# Autodesk Inventor assembly: Intake
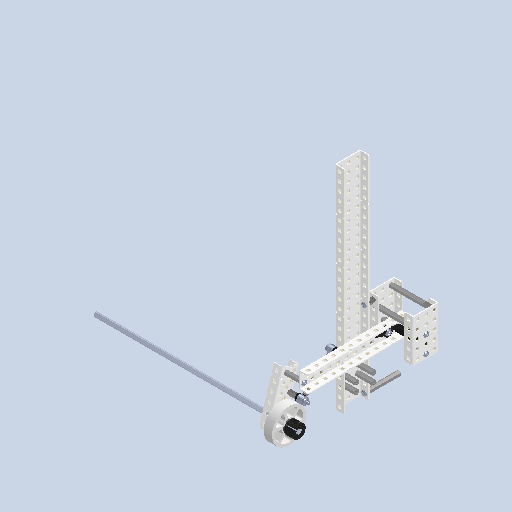
[picture p0: Inventor's stored thumbnail of the model, 512x512]
Saved by Autodesk Inventor 2023 (Build 270158000, 158)
## iProperties
Created: 2022-09-02
Part Number: Intake
Document SubType Name: Assembly
Designer: alex
Author: alex
## Documents named in this file (32)
- C:\Users\alex\Documents\GitHub\4067X_spin_up_cad\Mechanism\Intake.iam
- C:\Users\alex\Documents\GitHub\4067X_spin_up_cad\Library\Structure\C-Channels\Aluminum 1x3x1\Alu C 1x3x1x25.ipt
- C:\Users\alex\Documents\GitHub\4067X_spin_up_cad\Library\Structure\Standoff\Standoff 1.00.ipt
- C:\Users\alex\Documents\GitHub\4067X_spin_up_cad\Library\Structure\Standoff.ipt
- C:\Users\alex\Documents\GitHub\4067X_spin_up_cad\Library\Structure\Standoff\Standoff 2.00.ipt
- C:\Users\alex\Documents\GitHub\4067X_spin_up_cad\Library\Structure\Hardware\Screw Steel - Star\SScrew Star Smooth .290.ipt
- C:\Users\alex\Documents\GitHub\4067X_spin_up_cad\Library\Structure\Hardware\Screw Steel - Star.ipt
- C:\Users\alex\Documents\GitHub\4067X_spin_up_cad\Library\Structure\Standoff\Standoff .50.ipt
- C:\Users\alex\Documents\GitHub\4067X_spin_up_cad\Library\Structure\C-Channels\Aluminum 1x3x1\Alu C 1x3x1x5.ipt
- C:\Users\alex\Documents\GitHub\4067X_spin_up_cad\Library\Motion\Spacers\Spacer Nylon .375 OD.ipt
- C:\Users\alex\Documents\GitHub\4067X_spin_up_cad\Library\Motion\Spacers\Washer Teflon\TWasher .375 OD x .06250.ipt
- C:\Users\alex\Documents\GitHub\4067X_spin_up_cad\Library\Motion\Spacers\Washer Teflon.ipt
- C:\Users\alex\Documents\GitHub\4067X_spin_up_cad\Library\Structure\C-Channels\Aluminum 1x2x1\Alu C 1x2x1x6.ipt
- C:\Users\alex\Documents\GitHub\4067X_spin_up_cad\Library\Motion\Shaft HS\Shaft HS\Shaft HS 12.0 in.ipt
- C:\Users\alex\Documents\GitHub\4067X_spin_up_cad\Library\Motion\Shaft HS\Shaft HS.ipt
- C:\Users\alex\Documents\GitHub\4067X_spin_up_cad\Library\Motion\Spacers\Spacer Nylon .375 OD\NSpacer .375 OD x .125.ipt
- C:\Users\alex\Documents\GitHub\4067X_spin_up_cad\Library\Motion\Shaft Collar with Set Screw.ipt
- C:\Users\alex\Documents\GitHub\4067X_spin_up_cad\WithAdapter2Inch.iam
- C:\Users\alex\Documents\GitHub\4067X_spin_up_cad\Library\Motion\Shaft HS\HS Shaft Collar.ipt
- C:\Users\alex\Documents\GitHub\4067X_spin_up_cad\Library\Motion\Bearing Flat.ipt
- C:\Users\alex\Documents\GitHub\4067X_spin_up_cad\Library\Motion\Spacers\Spacer Nylon .375 OD\NSpacer .375 OD x .500.ipt
- C:\Users\alex\Documents\GitHub\4067X_spin_up_cad\Library\Motion\Spacers\Spacer Nylon .375 OD\NSpacer .375 OD x .375.ipt
- C:\Users\alex\Documents\GitHub\4067X_spin_up_cad\Library\Structure\Hardware\Screw Steel - Star\SScrew Star Smooth 1.250.ipt
- C:\Users\alex\Documents\GitHub\4067X_spin_up_cad\Library\Structure\Hardware\Nut Keps.ipt
- C:\Users\alex\Documents\GitHub\4067X_spin_up_cad\Library\Structure\Hardware\Screw Steel - Star\SScrew Star Smooth .625.ipt
- C:\Users\alex\Documents\GitHub\4067X_spin_up_cad\Library\Structure\Hardware\Screw Steel - Star\SScrew Star Threaded 2.500.ipt
- C:\Users\alex\Documents\GitHub\4067X_spin_up_cad\Library\Structure\C-Channels\Aluminum 1x2x1\Alu C 1x2x1x12.ipt
- C:\Users\alex\Documents\GitHub\4067X_spin_up_cad\Library\Motion\1-Post Bearing Flat Hex Retainer.ipt
- C:\Users\alex\Documents\GitHub\4067X_spin_up_cad\Library\Structure\Hardware\Screw Steel - Star\SScrew Star Smooth .375.ipt
- C:\Users\alex\Documents\GitHub\4067X_spin_up_cad\Library\Structure\Hardware\Nut Nylock.ipt
- C:\Users\alex\Documents\GitHub\4067X_spin_up_cad\Library\Structure\Hardware\Screw Steel - Star\SScrew Star Smooth .500.ipt
- C:\Users\alex\Documents\GitHub\4067X_spin_up_cad\Library\Structure\Hardware\Nut Thin Nylock.ipt
## Components (57 placed, 26 different names)
1. Alu C 1x3x1x25:1 — Insert:1, Insert:2, Insert:3, Insert:4, Insert:5, Insert:7, Insert:8, Insert:9, Insert:10, Insert:11, Insert:12, Insert:13, Insert:14, Insert:19
2. Standoff 1.00:1 — Insert:1
3. Standoff 1.00:2 — Insert:2
4. Standoff 1.00:3 — Insert:3
5. Standoff 1.00:4 — Insert:4
6. Standoff 2.00:5 — Insert:5
7. SScrew Star Smooth .290:1 — Insert:7
8. SScrew Star Smooth .290:2 — Insert:8
9. SScrew Star Smooth .290:3 — Insert:9
10. SScrew Star Smooth .290:4 — Insert:10
11. SScrew Star Smooth .290:5 — Insert:11
12. SScrew Star Smooth .290:6 — Insert:12
13. Standoff .50:6 — Insert:13, Insert:16
14. Alu C 1x3x1x5:1 — Insert:15, Insert:16, Insert:17, Insert:20, Insert:21, Insert:22, Insert:68, Insert:69, Insert:81, Insert:86
15. Standoff .50:7 — Insert:14, Insert:15
16. Standoff 2.00:8 — Insert:17, Insert:105
17. SScrew Star Smooth .290:7 — Insert:19
18. SScrew Star Smooth .290:8 — Insert:20
19. SScrew Star Smooth .290:9 — Insert:21
20. SScrew Star Smooth .290:10 — Insert:22
21. Alu C 1x2x1x6:1 — Mate:2, Mate:3, Insert:39, Insert:40, Mate:11, Insert:48, Insert:50
22. Shaft HS 12.0 in:1 — Mate:2, Mate:5, Mate:6, Mate:9, Mate:10, Flush:1
23. NSpacer .375 OD x .125:1 — Insert:34, Insert:73
24. Shaft Collar with Set Screw:1 — Insert:34, Mate:4, Mate:7, Insert:53
25. Shaft Collar with Set Screw:2 — Mate:3, Mate:4, Insert:35, Insert:49
26. WithAdapter2Inch:1 [sub-assembly] — Mate:5, Mate:6, Mate:8, Mate:11
27. Standoff 2.00:12 — Insert:35, Mate:7
28. Standoff .50:14 — Insert:38, Insert:39
29. NSpacer .375 OD x .125:2 — Insert:38
30. Standoff 1.00:15 — Insert:40, Insert:71
31. HS Shaft Collar:1 — Mate:8, Mate:9, Mate:10, Flush:1
32. SScrew Star Smooth 1.250:13 — Insert:48
33. Nut Keps:1 — Insert:49
34. SScrew Star Smooth .290:14 — Insert:50
35. SScrew Star Smooth .290:15 — Insert:72
36. SScrew Star Smooth .625:16 — Insert:74
37. Nut Keps:2 — Insert:53
38. SScrew Star Smooth .290:23 — Insert:68
39. Standoff 2.00:18 — Insert:69, Insert:106
40. Alu C 1x2x1x12:1 — Insert:71, Insert:72, Insert:73, Insert:74, Insert:83, Insert:102, Mate:12, Insert:103
41. Standoff .50:21 — Insert:81, Insert:82
42. TWasher .375 OD x .06250:1 — Insert:82, Insert:83
43. SScrew Star Threaded 2.500:25 — Insert:86
44. NSpacer .375 OD x .500:6 — Insert:111
45. 1-Post Bearing Flat Hex Retainer:1 — Insert:102, Mate:12, Insert:104
46. SScrew Star Smooth .375:30 — Insert:103
47. Nut Nylock:1 — Insert:104
48. Alu C 1x3x1x5:2 — Insert:107, Insert:108, Insert:109, Insert:110, Insert:113, Insert:114
49. Standoff .50:22 — Insert:105, Insert:107
50. Standoff .50:23 — Insert:106, Insert:108
51. Bearing Flat:3 — Insert:109, Insert:110, Insert:115, Insert:116
52. NSpacer .375 OD x .500:7 — Insert:111, Insert:112
53. NSpacer .375 OD x .375:8 — Insert:112
54. SScrew Star Smooth .500:31 — Insert:113
55. SScrew Star Smooth .500:32 — Insert:114
56. Nut Thin Nylock:1 — Insert:115
57. Nut Thin Nylock:2 — Insert:116
## Relationships (66: Insert 54, Mate 11, Flush 1)
- Insert:1: Alu C 1x3x1x25:1 ↔ Standoff 1.00:1
- Insert:2: Alu C 1x3x1x25:1 ↔ Standoff 1.00:2
- Insert:3: Alu C 1x3x1x25:1 ↔ Standoff 1.00:3
- Insert:4: Alu C 1x3x1x25:1 ↔ Standoff 1.00:4
- Insert:5: Alu C 1x3x1x25:1 ↔ Standoff 2.00:5
- Insert:7: Alu C 1x3x1x25:1 ↔ SScrew Star Smooth .290:1
- Insert:8: Alu C 1x3x1x25:1 ↔ SScrew Star Smooth .290:2
- Insert:9: Alu C 1x3x1x25:1 ↔ SScrew Star Smooth .290:3
- Insert:10: Alu C 1x3x1x25:1 ↔ SScrew Star Smooth .290:4
- Insert:11: Alu C 1x3x1x25:1 ↔ SScrew Star Smooth .290:5
- Insert:12: Alu C 1x3x1x25:1 ↔ SScrew Star Smooth .290:6
- Insert:13: Alu C 1x3x1x25:1 ↔ Standoff .50:6
- Insert:14: Alu C 1x3x1x25:1 ↔ Standoff .50:7
- Insert:15: Alu C 1x3x1x5:1 ↔ Standoff .50:7
- Insert:16: Standoff .50:6 ↔ Alu C 1x3x1x5:1
- Insert:17: Alu C 1x3x1x5:1 ↔ Standoff 2.00:8
- Insert:19: Alu C 1x3x1x25:1 ↔ SScrew Star Smooth .290:7
- Insert:20: Alu C 1x3x1x5:1 ↔ SScrew Star Smooth .290:8
- Insert:21: Alu C 1x3x1x5:1 ↔ SScrew Star Smooth .290:9
- Insert:22: Alu C 1x3x1x5:1 ↔ SScrew Star Smooth .290:10
- Mate:2: Alu C 1x2x1x6:1 ↔ Shaft HS 12.0 in:1
- Insert:34: NSpacer .375 OD x .125:1 ↔ Shaft Collar with Set Screw:1
- Mate:3: Alu C 1x2x1x6:1 ↔ Shaft Collar with Set Screw:2
- Mate:4: Shaft Collar with Set Screw:1 ↔ Shaft Collar with Set Screw:2
- Mate:5: Shaft HS 12.0 in:1 ↔ WithAdapter2Inch:1
- Mate:6: Shaft HS 12.0 in:1 ↔ WithAdapter2Inch:1
- Insert:35 (-0.3556 mm): Shaft Collar with Set Screw:2 ↔ Standoff 2.00:12
- Mate:7 (-0.3556 mm): Shaft Collar with Set Screw:1 ↔ Standoff 2.00:12
- Insert:38: Standoff .50:14 ↔ NSpacer .375 OD x .125:2
- Insert:39: Alu C 1x2x1x6:1 ↔ Standoff .50:14
- Insert:40: Alu C 1x2x1x6:1 ↔ Standoff 1.00:15
- Mate:8: WithAdapter2Inch:1 ↔ HS Shaft Collar:1
- Mate:9: Shaft HS 12.0 in:1 ↔ HS Shaft Collar:1
- Mate:10: Shaft HS 12.0 in:1 ↔ HS Shaft Collar:1
- Flush:1 (-0.3556 mm): Shaft HS 12.0 in:1 ↔ HS Shaft Collar:1
- Mate:11: Alu C 1x2x1x6:1 ↔ WithAdapter2Inch:1
- Insert:48: Alu C 1x2x1x6:1 ↔ SScrew Star Smooth 1.250:13
- Insert:49: Shaft Collar with Set Screw:2 ↔ Nut Keps:1
- Insert:50: Alu C 1x2x1x6:1 ↔ SScrew Star Smooth .290:14
- Insert:53: Shaft Collar with Set Screw:1 ↔ Nut Keps:2
- Insert:68: Alu C 1x3x1x5:1 ↔ SScrew Star Smooth .290:23
- Insert:69: Alu C 1x3x1x5:1 ↔ Standoff 2.00:18
- Insert:71: Standoff 1.00:15 ↔ Alu C 1x2x1x12:1
- Insert:72: SScrew Star Smooth .290:15 ↔ Alu C 1x2x1x12:1
- Insert:73: NSpacer .375 OD x .125:1 ↔ Alu C 1x2x1x12:1
- Insert:74: SScrew Star Smooth .625:16 ↔ Alu C 1x2x1x12:1
- Insert:81: Alu C 1x3x1x5:1 ↔ Standoff .50:21
- Insert:82: Standoff .50:21 ↔ TWasher .375 OD x .06250:1
- Insert:83: Alu C 1x2x1x12:1 ↔ TWasher .375 OD x .06250:1
- Insert:86: Alu C 1x3x1x5:1 ↔ SScrew Star Threaded 2.500:25
- Insert:102: Alu C 1x2x1x12:1 ↔ 1-Post Bearing Flat Hex Retainer:1
- Mate:12: Alu C 1x2x1x12:1 ↔ 1-Post Bearing Flat Hex Retainer:1
- Insert:103: Alu C 1x2x1x12:1 ↔ SScrew Star Smooth .375:30
- Insert:104: 1-Post Bearing Flat Hex Retainer:1 ↔ Nut Nylock:1
- Insert:105: Standoff 2.00:8 ↔ Standoff .50:22
- Insert:106: Standoff 2.00:18 ↔ Standoff .50:23
- Insert:107: Alu C 1x3x1x5:2 ↔ Standoff .50:22
- Insert:108: Alu C 1x3x1x5:2 ↔ Standoff .50:23
- Insert:109: Alu C 1x3x1x5:2 ↔ Bearing Flat:3
- Insert:110: Alu C 1x3x1x5:2 ↔ Bearing Flat:3
- Insert:111: NSpacer .375 OD x .500:6 ↔ NSpacer .375 OD x .500:7
- Insert:112: NSpacer .375 OD x .500:7 ↔ NSpacer .375 OD x .375:8
- Insert:113: Alu C 1x3x1x5:2 ↔ SScrew Star Smooth .500:31
- Insert:114: Alu C 1x3x1x5:2 ↔ SScrew Star Smooth .500:32
- Insert:115: Bearing Flat:3 ↔ Nut Thin Nylock:1
- Insert:116: Bearing Flat:3 ↔ Nut Thin Nylock:2
